# Autodesk Inventor assembly: ForLaserCut
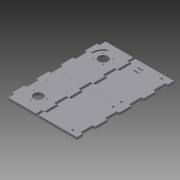
[picture p0: Inventor's stored thumbnail of the model, 180x180]
Saved by Autodesk Inventor 2015 (Build 190159000, 159)
## iProperties
Created: 2017-03-15
Part Number: ForLaserCut
Document SubType Name: Assembly
Designer: Ernest
Author: Ernest
## Documents named in this file (5)
- C:\Users\Ernest\Documents\Capstone-Project\doc\CAD\LowLevel_Rev3\EE_base\ForLaserCut.iam
- C:\Users\Ernest\Documents\Capstone-Project\doc\CAD\LowLevel_Rev3\EE_base\bottom.ipt
- C:\Users\Ernest\Documents\Capstone-Project\doc\CAD\LowLevel_Rev3\EE_base\SideLeft.ipt
- C:\Users\Ernest\Documents\Capstone-Project\doc\CAD\LowLevel_Rev3\EE_base\SideRight.ipt
- C:\Users\Ernest\Documents\Capstone-Project\doc\CAD\LowLevel_Rev3\EE_base\top.ipt
## Components (4 placed, 4 different names)
1. bottom:1 — Flush:1, Flush:2, Flush:3, Flush:5, Mate:2, Flush:7
2. SideLeft:1 — Flush:2, Mate:1, Flush:4, Angle:1, Mate:3, Flush:6
3. SideRight:1 — Flush:3, Flush:4, Flush:7
4. top:1 — Flush:1, Flush:5, Angle:1, Mate:2, Mate:3, Flush:6
## Relationships (11: Flush 7, Mate 3, Angle 1)
- Flush:1: bottom:1 ↔ top:1
- Flush:2: bottom:1 ↔ SideLeft:1
- Flush:3: bottom:1 ↔ SideRight:1
- Mate:1: SideLeft:1
- Flush:4: SideLeft:1 ↔ SideRight:1
- Flush:5: bottom:1 ↔ top:1
- Angle:1 (0 deg): SideLeft:1 ↔ top:1
- Mate:2 (0.2 mm): bottom:1 ↔ top:1
- Mate:3 (0.2 mm): SideLeft:1 ↔ top:1
- Flush:6: SideLeft:1 ↔ top:1
- Flush:7: bottom:1 ↔ SideRight:1
